# Autodesk Inventor assembly: Assembly3
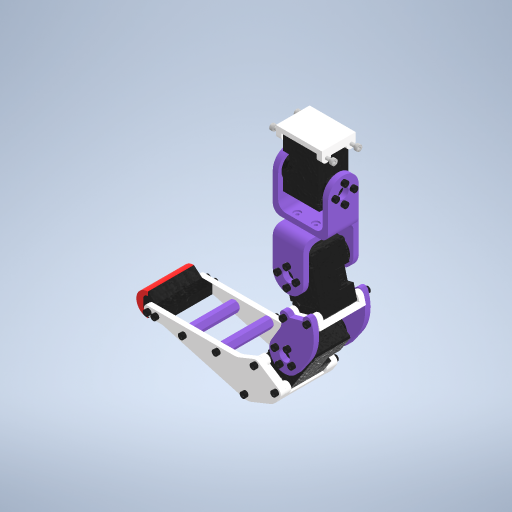
[picture p0: Inventor's stored thumbnail of the model, 512x512]
Saved by Autodesk Inventor 2024 (Build 280153000, 153)
## iProperties
Created: 2024-06-02
Part Number: Assembly3
Document SubType Name: Assembly
Designer: Hemant
Author: Hemant
## iProperties of the stored document DC15_A01_CASE_M_DUMMY.ipt
Created: 2020-07-27
Part Number: DC15_A01_CASE_M_DUMMY
Material: Generic
Description: NOT SPECIFIED
Document SubType Name: Modeling
Designer: Hemant
Mass: 9.54609 g
Surface Area: 36.4084 cm^2
Volume: 9.54609 cm^3
Density: 1 g/cm^3
Appearance: Default
Author: Hemant
Revision Number: 7LAST_VERSION
## iProperties of the stored document PHS_1_7X20_5_DC10.ipt
Created: 2020-07-27
Part Number: PHS_1_7X20_5_DC10
Material: Generic
Description: NOT SPECIFIED
Document SubType Name: Modeling
Designer: Hemant
Density: 1 g/cm^3
Appearance: Default
Author: Hemant
Revision Number: 3LAST_VERSION
## iProperties of the stored document DC15_A01_HORN_DUMMY.ipt
Created: 2020-07-27
Part Number: DC15_A01_HORN_DUMMY
Material: Generic
Description: NOT SPECIFIED
Document SubType Name: Modeling
Designer: Hemant
Density: 1 g/cm^3
Appearance: Default
Author: Hemant
Revision Number: 17LAST_VERSION
## iProperties of the stored document BTS2_M2_6X8.ipt
Created: 2020-07-27
Part Number: BTS2_M2_6X8
Material: Generic
Description: NOT SPECIFIED
Document SubType Name: Modeling
Designer: Hemant
Density: 1 g/cm^3
Appearance: Default
Author: Hemant
Revision Number: 5LAST_VERSION
## iProperties of the stored document DC15_A01_HORN_IDLE2_DUMMY.ipt
Created: 2020-07-27
Part Number: DC15_A01_HORN_IDLE2_DUMMY
Material: Generic
Description: NOT SPECIFIED
Document SubType Name: Modeling
Designer: Hemant
Density: 1 g/cm^3
Appearance: Default
Author: Hemant
Revision Number: 2LAST_VERSION
## iProperties of the stored document XL,XC-330.iam
Created: 2020-07-27
Part Number: DC15_A01_DUMMY_ASSY_IDLE_ASM
Document SubType Name: Assembly
Designer: Hemant
Sending System: CREO PARAMETRIC BY PTC INC, 2019224
Preprocessor: CREO PARAMETRIC BY PTC INC, 2019224
Title: DC15_A01_DUMMY_ASSY_IDLE_ASM
Author: yunever
Revision Number: 9LAST_VERSION
## iProperties of the stored document DC15_A01_CASE_F_DUMMY.ipt
Created: 2020-07-27
Part Number: DC15_A01_CASE_F_DUMMY
Material: Generic
Description: NOT SPECIFIED
Document SubType Name: Modeling
Designer: Hemant
Density: 1 g/cm^3
Appearance: Default
Author: Hemant
Revision Number: 5LAST_VERSION
## iProperties of the stored document DC15_A01_IDLE_CAP_DUMMY.ipt
Created: 2020-07-27
Part Number: DC15_A01_IDLE_CAP_DUMMY
Material: Generic
Description: NOT SPECIFIED
Document SubType Name: Modeling
Designer: Hemant
Density: 1 g/cm^3
Appearance: Default
Author: Hemant
Revision Number: 2LAST_VERSION
## iProperties of the stored document DC15_A01_CASE_B_DUMMY.ipt
Created: 2020-07-27
Part Number: DC15_A01_CASE_B_DUMMY
Material: Generic
Description: NOT SPECIFIED
Document SubType Name: Modeling
Designer: Hemant
Density: 1 g/cm^3
Appearance: Default
Mass: 2.59492 g
Surface Area: 23.2234 cm^2
Volume: 2.59492 cm^3
Author: Hemant
Revision Number: 8LAST_VERSION
## iProperties of the stored document B3B-EH.ipt
Created: 2020-07-27
Part Number: B3B-EH
Material: Generic
Description: NOT SPECIFIED
Document SubType Name: Modeling
Designer: Hemant
Density: 1 g/cm^3
Appearance: Default
Author: Hemant
Revision Number: 2LAST_VERSION
## iProperties of the stored document DC15_A01_LED_CAP2_DUMMY.ipt
Created: 2020-07-27
Part Number: DC15_A01_LED_CAP2_DUMMY
Material: Generic
Description: NOT SPECIFIED
Document SubType Name: Modeling
Designer: Hemant
Density: 1 g/cm^3
Appearance: Default
Author: Hemant
Revision Number: 3LAST_VERSION
## Documents named in this file (22)
- C:\Users\Hemant\Desktop\Studies\MS Proj\V1\Leg_assembly_V2.iam
- **C:\Users\Hemant\Desktop\Studies\MS Proj\V1\Leg_assembly_V2.iam*LocalDocs*xAaaaaedaAaaaaaaaAaaaqztbHd*XL,XC-330.iam
- C:\Users\Hemant\Desktop\Studies\MS Proj\V1\Motor_Bracket.ipt
- C:\Users\Hemant\Desktop\Studies\MS Proj\V1\Motor_Base.ipt
- C:\Users\Hemant\Desktop\Studies\MS Proj\V1\Tibia_Femur_Connect.ipt
- C:\Users\Hemant\Desktop\Studies\MS Proj\V1\Standoff.ipt
- C:\Users\Hemant\Desktop\Studies\MS Proj\V1\socket head cap screw_iso_ISO 4762 M2 x 5 --- 5S.ipt
- C:\Users\Hemant\Desktop\Studies\MS Proj\V1\Tibia_V2.ipt
- C:\Users\Hemant\Desktop\Studies\MS Proj\V1\Foot_V1.ipt
- C:\Users\Hemant\Desktop\Studies\MS Proj\V1\TPU_FootGrip.ipt
- C:\Users\Hemant\Desktop\Studies\MS Proj\XL,XC-330.stp
- **C:\Users\Hemant\Desktop\Studies\MS Proj\V1\Assembly3.iam*LocalDocs*xAaaaaedaAaaaaaaaAaaaqzd4Uh*DC15_A01_CASE_M_DUMMY.ipt
- **C:\Users\Hemant\Desktop\Studies\MS Proj\V1\Assembly3.iam*LocalDocs*xAaaaa1caAaaaaaaaAaaaaeqcGe*PHS_1_7X20_5_DC10.ipt
- **C:\Users\Hemant\Desktop\Studies\MS Proj\V1\Assembly3.iam*LocalDocs*xAaaaa0caAaaaaaaaAaaaan2dPg*DC15_A01_HORN_DUMMY.ipt
- **C:\Users\Hemant\Desktop\Studies\MS Proj\V1\Assembly3.iam*LocalDocs*xAaaaaabaAaaaaaaaAaaaag1aQf*BTS2_M2_6X8.ipt
- **C:\Users\Hemant\Desktop\Studies\MS Proj\V1\Assembly3.iam*LocalDocs*xAaaaalaaAaaaaaaaAaaaqc1fQc*DC15_A01_HORN_IDLE2_DUMMY.ipt
- **C:\Users\Hemant\Desktop\Studies\MS Proj\V1\Assembly3.iam*LocalDocs*xAaaaaedaAaaaaaaaAaaaqztbHd*XL,XC-330.iam
- **C:\Users\Hemant\Desktop\Studies\MS Proj\V1\Assembly3.iam*LocalDocs*xAaaaqebaAaaaaaaaAaaaamr1Rh*DC15_A01_CASE_F_DUMMY.ipt
- **C:\Users\Hemant\Desktop\Studies\MS Proj\V1\Assembly3.iam*LocalDocs*xAaaaqhbaAaaaaaaaAaaaqpykVc*DC15_A01_CASE_B_DUMMY.ipt
- **C:\Users\Hemant\Desktop\Studies\MS Proj\V1\Assembly3.iam*LocalDocs*xAaaaqkcaAaaaaaaaAaaaa1g0If*DC15_A01_LED_CAP2_DUMMY.ipt
- **C:\Users\Hemant\Desktop\Studies\MS Proj\V1\Assembly3.iam*LocalDocs*xAaaaazdaAaaaaaaaAaaaawueFb*DC15_A01_IDLE_CAP_DUMMY.ipt
- **C:\Users\Hemant\Desktop\Studies\MS Proj\V1\Assembly3.iam*LocalDocs*xAaaaqfcaAaaaaaaaAaaaawcvTg*B3B-EH.ipt
## Components (59 placed, 9 different names)
1. XL,XC-330:1 [sub-assembly] — Mate:1, Mate:2_Supress, Mate:3, Mate:4, Mate:5, Mate:6, Angle:3_Supress
2. Motor_Bracket:2 — Mate:1, Mate:2_Supress, Mate:3, Mate:7, Mate:8, Mate:9, Mate:60, Mate:61, Mate:62, Mate:63, Mate:78, Mate:79, Mate:80, Mate:81, Mate:88, Mate:89, Mate:90, Mate:91, Mate:100, Mate:101, Mate:102, Mate:103
3. Motor_Base:1 — Mate:4, Mate:5, Mate:6, Mate:10, Mate:11, Mate:12, Mate:13, Mate:14, Mate:15
4. Motor_Bracket:3 — Mate:7, Mate:8, Mate:9, Mate:16, Mate:17, Mate:26_Supress, Angle:3_Supress, Mate:64, Mate:65, Mate:66, Mate:67, Mate:74, Mate:75, Mate:76, Mate:77
5. Tibia_Femur_Connect:1 — Mate:11, Mate:14, Mate:15, Mate:19, Mate:92, Mate:93, Mate:94, Mate:95, Mate:96, Mate:97, Mate:98, Mate:99, Mate:108, Mate:109, Mate:110, Mate:111
6. Tibia_Femur_Connect:2 — Mate:10, Mate:12, Mate:13, Mate:18, Angle:2_Supress, Mate:56, Mate:57, Mate:58, Mate:59, Mate:70, Mate:71, Mate:72, Mate:73, Mate:84, Mate:85, Mate:86, Mate:87
7. XL,XC-330:2 [sub-assembly] — Mate:16, Mate:17, Angle:1, Mate:26_Supress, Mate:33, Mate:34, Mate:35
8. XL,XC-330:3 [sub-assembly] — Mate:18, Mate:19, Angle:2_Supress, Mate:20, Mate:21, Mate:22
9. Motor_Base:2 — Mate:20, Mate:21, Mate:22, Mate:122, Mate:123, Mate:124, Mate:127, Mate:128, Mate:129
10. Motor_Base:3 — Mate:33, Mate:34, Mate:35, Mate:68, Mate:69, Mate:82, Mate:83, Mate:116, Mate:117, Mate:120, Mate:121, Angle:4_Supress
11. Standoff:1 — Mate:130, Mate:131
12. socket head cap screw_iso_ISO 4762 M2 x 5 --- 5S:2 — Mate:144, Mate:151
13. socket head cap screw_iso_ISO 4762 M2 x 5 --- 5S:3 — Mate:145, Mate:154
14. socket head cap screw_iso_ISO 4762 M2 x 5 --- 5S:4 — Mate:146, Mate:152
15. socket head cap screw_iso_ISO 4762 M2 x 5 --- 5S:5 — Mate:140, Mate:166
16. socket head cap screw_iso_ISO 4762 M2 x 5 --- 5S:6 — Mate:139, Mate:167
17. socket head cap screw_iso_ISO 4762 M2 x 5 --- 5S:7 — Mate:84, Mate:87
18. socket head cap screw_iso_ISO 4762 M2 x 5 --- 5S:8 — Mate:85, Mate:86
19. socket head cap screw_iso_ISO 4762 M2 x 5 --- 5S:9 — Mate:58, Mate:72
20. socket head cap screw_iso_ISO 4762 M2 x 5 --- 5S:10 — Mate:61, Mate:81
21. socket head cap screw_iso_ISO 4762 M2 x 5 --- 5S:11 — Mate:60, Mate:78
22. socket head cap screw_iso_ISO 4762 M2 x 5 --- 5S:12 — Mate:57, Mate:73
23. socket head cap screw_iso_ISO 4762 M2 x 5 --- 5S:13 — Mate:64, Mate:77
24. socket head cap screw_iso_ISO 4762 M2 x 5 --- 5S:14 — Mate:65, Mate:74
25. socket head cap screw_iso_ISO 4762 M2 x 5 --- 5S:15 — Mate:90, Mate:101
26. socket head cap screw_iso_ISO 4762 M2 x 5 --- 5S:16 — Mate:91, Mate:102
27. socket head cap screw_iso_ISO 4762 M2 x 5 --- 5S:17 — Mate:62, Mate:79
28. socket head cap screw_iso_ISO 4762 M2 x 5 --- 5S:18 — Mate:68, Mate:82
29. socket head cap screw_iso_ISO 4762 M2 x 5 --- 5S:19 — Mate:69, Mate:83
30. socket head cap screw_iso_ISO 4762 M2 x 5 --- 5S:20 — Mate:63, Mate:80
31. socket head cap screw_iso_ISO 4762 M2 x 5 --- 5S:21 — Mate:66, Mate:76
32. socket head cap screw_iso_ISO 4762 M2 x 5 --- 5S:22 — Mate:67, Mate:75
33. socket head cap screw_iso_ISO 4762 M2 x 5 --- 5S:23 — Mate:88, Mate:100
34. socket head cap screw_iso_ISO 4762 M2 x 5 --- 5S:24 — Mate:89, Mate:103
35. socket head cap screw_iso_ISO 4762 M2 x 5 --- 5S:25 — Mate:92, Mate:99
36. socket head cap screw_iso_ISO 4762 M2 x 5 --- 5S:26 — Mate:93, Mate:98
37. socket head cap screw_iso_ISO 4762 M2 x 5 --- 5S:27 — Mate:94, Mate:97
38. socket head cap screw_iso_ISO 4762 M2 x 5 --- 5S:28 — Mate:95, Mate:96
39. socket head cap screw_iso_ISO 4762 M2 x 5 --- 5S:30 — Mate:156, Mate:159
40. socket head cap screw_iso_ISO 4762 M2 x 5 --- 5S:31 — Mate:56, Mate:71
41. socket head cap screw_iso_ISO 4762 M2 x 5 --- 5S:32 — Mate:59, Mate:70
42. socket head cap screw_iso_ISO 4762 M2 x 5 --- 5S:35 — Mate:116, Mate:120
43. socket head cap screw_iso_ISO 4762 M2 x 5 --- 5S:36 — Mate:117, Mate:121
44. socket head cap screw_iso_ISO 4762 M2 x 5 --- 5S:37 — Mate:142, Mate:169
45. socket head cap screw_iso_ISO 4762 M2 x 5 --- 5S:38 — Mate:141, Mate:168
46. socket head cap screw_iso_ISO 4762 M2 x 5 --- 5S:39 — Mate:109, Mate:111
47. socket head cap screw_iso_ISO 4762 M2 x 5 --- 5S:40 — Mate:108, Mate:110
48. Tibia_V2:1 — Mate:127, Mate:128, Mate:129, Mate:131, Angle:4_Supress, Mate:137, Mate:139, Mate:140, Mate:144, Mate:145, Mate:146, Mate:151, Mate:152, Mate:154, Mate:166, Mate:167, Mate:171, Mate:172, Mate:178, Mate:179, Mate:180, Mate:181, Angle:5
49. Tibia_V2:2 — Mate:122, Mate:123, Mate:124, Mate:130, Mate:136, Mate:138, Mate:141, Mate:142, Mate:156, Mate:159, Mate:160, Mate:161, Mate:164, Mate:165, Mate:168, Mate:169, Mate:170, Mate:173, Mate:174, Mate:175, Mate:176, Mate:177
50. Foot_V1:1 — Mate:136, Mate:137, Mate:138, Mate:148, Mate:149, Mate:150
51. TPU_FootGrip:1 — Mate:148, Mate:149, Mate:150
52. socket head cap screw_iso_ISO 4762 M2 x 5 --- 5S:41 — Mate:160, Mate:164
53. socket head cap screw_iso_ISO 4762 M2 x 5 --- 5S:42 — Mate:161, Mate:165
54. Standoff:2 — Mate:170, Mate:171, Angle:5
55. socket head cap screw_iso_ISO 4762 M2 x 5 --- 5S:43 — Mate:175, Mate:177
56. socket head cap screw_iso_ISO 4762 M2 x 5 --- 5S:44 — Mate:179, Mate:181
57. Standoff:3 — Mate:172, Mate:173
58. socket head cap screw_iso_ISO 4762 M2 x 5 --- 5S:45 — Mate:174, Mate:176
59. socket head cap screw_iso_ISO 4762 M2 x 5 --- 5S:46 — Mate:178, Mate:180
## Relationships (133: Mate 128, Angle 5)
- Mate:1: XL,XC-330:1 ↔ Motor_Bracket:2
- Mate:2_Supress: XL,XC-330:1 ↔ Motor_Bracket:2
- Mate:3: XL,XC-330:1 ↔ Motor_Bracket:2
- Mate:4: XL,XC-330:1 ↔ Motor_Base:1
- Mate:5: XL,XC-330:1 ↔ Motor_Base:1
- Mate:6: XL,XC-330:1 ↔ Motor_Base:1
- Mate:7: Motor_Bracket:2 ↔ Motor_Bracket:3
- Mate:8: Motor_Bracket:2 ↔ Motor_Bracket:3
- Mate:9: Motor_Bracket:2 ↔ Motor_Bracket:3
- Mate:10: Motor_Base:1 ↔ Tibia_Femur_Connect:2
- Mate:11: Motor_Base:1 ↔ Tibia_Femur_Connect:1
- Mate:12: Motor_Base:1 ↔ Tibia_Femur_Connect:2
- Mate:13: Motor_Base:1 ↔ Tibia_Femur_Connect:2
- Mate:14: Motor_Base:1 ↔ Tibia_Femur_Connect:1
- Mate:15: Motor_Base:1 ↔ Tibia_Femur_Connect:1
- Mate:16: Motor_Bracket:3 ↔ XL,XC-330:2
- Mate:17: Motor_Bracket:3 ↔ XL,XC-330:2
- Angle:1 (0 deg): XL,XC-330:2
- Mate:18: Tibia_Femur_Connect:2 ↔ XL,XC-330:3
- Mate:19 (0.5 mm): Tibia_Femur_Connect:1 ↔ XL,XC-330:3
- Angle:2_Supress (0 deg): Tibia_Femur_Connect:2 ↔ XL,XC-330:3
- Mate:20: XL,XC-330:3 ↔ Motor_Base:2
- Mate:21: XL,XC-330:3 ↔ Motor_Base:2
- Mate:22: XL,XC-330:3 ↔ Motor_Base:2
- Mate:26_Supress: Motor_Bracket:3 ↔ XL,XC-330:2
- Angle:3_Supress (0 deg): XL,XC-330:1 ↔ Motor_Bracket:3
- Mate:33: XL,XC-330:2 ↔ Motor_Base:3
- Mate:34: XL,XC-330:2 ↔ Motor_Base:3
- Mate:35: XL,XC-330:2 ↔ Motor_Base:3
- Mate:56: Tibia_Femur_Connect:2 ↔ socket head cap screw_iso_ISO 4762 M2 x 5 --- 5S:31
- Mate:57: Tibia_Femur_Connect:2 ↔ socket head cap screw_iso_ISO 4762 M2 x 5 --- 5S:12
- Mate:58: Tibia_Femur_Connect:2 ↔ socket head cap screw_iso_ISO 4762 M2 x 5 --- 5S:9
- Mate:59: Tibia_Femur_Connect:2 ↔ socket head cap screw_iso_ISO 4762 M2 x 5 --- 5S:32
- Mate:60: Motor_Bracket:2 ↔ socket head cap screw_iso_ISO 4762 M2 x 5 --- 5S:11
- Mate:61: Motor_Bracket:2 ↔ socket head cap screw_iso_ISO 4762 M2 x 5 --- 5S:10
- Mate:62: Motor_Bracket:2 ↔ socket head cap screw_iso_ISO 4762 M2 x 5 --- 5S:17
- Mate:63: Motor_Bracket:2 ↔ socket head cap screw_iso_ISO 4762 M2 x 5 --- 5S:20
- Mate:64: Motor_Bracket:3 ↔ socket head cap screw_iso_ISO 4762 M2 x 5 --- 5S:13
- Mate:65: Motor_Bracket:3 ↔ socket head cap screw_iso_ISO 4762 M2 x 5 --- 5S:14
- Mate:66: Motor_Bracket:3 ↔ socket head cap screw_iso_ISO 4762 M2 x 5 --- 5S:21
- Mate:67: Motor_Bracket:3 ↔ socket head cap screw_iso_ISO 4762 M2 x 5 --- 5S:22
- Mate:68 (3.5 mm): Motor_Base:3 ↔ socket head cap screw_iso_ISO 4762 M2 x 5 --- 5S:18
- Mate:69 (3.5 mm): Motor_Base:3 ↔ socket head cap screw_iso_ISO 4762 M2 x 5 --- 5S:19
- Mate:70: Tibia_Femur_Connect:2 ↔ socket head cap screw_iso_ISO 4762 M2 x 5 --- 5S:32
- Mate:71: Tibia_Femur_Connect:2 ↔ socket head cap screw_iso_ISO 4762 M2 x 5 --- 5S:31
- Mate:72: Tibia_Femur_Connect:2 ↔ socket head cap screw_iso_ISO 4762 M2 x 5 --- 5S:9
- Mate:73: Tibia_Femur_Connect:2 ↔ socket head cap screw_iso_ISO 4762 M2 x 5 --- 5S:12
- Mate:74: Motor_Bracket:3 ↔ socket head cap screw_iso_ISO 4762 M2 x 5 --- 5S:14
- Mate:75: Motor_Bracket:3 ↔ socket head cap screw_iso_ISO 4762 M2 x 5 --- 5S:22
- Mate:76: Motor_Bracket:3 ↔ socket head cap screw_iso_ISO 4762 M2 x 5 --- 5S:21
- Mate:77: Motor_Bracket:3 ↔ socket head cap screw_iso_ISO 4762 M2 x 5 --- 5S:13
- Mate:78: Motor_Bracket:2 ↔ socket head cap screw_iso_ISO 4762 M2 x 5 --- 5S:11
- Mate:79: Motor_Bracket:2 ↔ socket head cap screw_iso_ISO 4762 M2 x 5 --- 5S:17
- Mate:80: Motor_Bracket:2 ↔ socket head cap screw_iso_ISO 4762 M2 x 5 --- 5S:20
- Mate:81: Motor_Bracket:2 ↔ socket head cap screw_iso_ISO 4762 M2 x 5 --- 5S:10
- Mate:82: Motor_Base:3 ↔ socket head cap screw_iso_ISO 4762 M2 x 5 --- 5S:18
- Mate:83: Motor_Base:3 ↔ socket head cap screw_iso_ISO 4762 M2 x 5 --- 5S:19
- Mate:84: Tibia_Femur_Connect:2 ↔ socket head cap screw_iso_ISO 4762 M2 x 5 --- 5S:7
- Mate:85: Tibia_Femur_Connect:2 ↔ socket head cap screw_iso_ISO 4762 M2 x 5 --- 5S:8
- Mate:86: Tibia_Femur_Connect:2 ↔ socket head cap screw_iso_ISO 4762 M2 x 5 --- 5S:8
- Mate:87: Tibia_Femur_Connect:2 ↔ socket head cap screw_iso_ISO 4762 M2 x 5 --- 5S:7
- Mate:88: Motor_Bracket:2 ↔ socket head cap screw_iso_ISO 4762 M2 x 5 --- 5S:23
- Mate:89: Motor_Bracket:2 ↔ socket head cap screw_iso_ISO 4762 M2 x 5 --- 5S:24
- Mate:90: Motor_Bracket:2 ↔ socket head cap screw_iso_ISO 4762 M2 x 5 --- 5S:15
- Mate:91: Motor_Bracket:2 ↔ socket head cap screw_iso_ISO 4762 M2 x 5 --- 5S:16
- Mate:92: Tibia_Femur_Connect:1 ↔ socket head cap screw_iso_ISO 4762 M2 x 5 --- 5S:25
- Mate:93: Tibia_Femur_Connect:1 ↔ socket head cap screw_iso_ISO 4762 M2 x 5 --- 5S:26
- Mate:94: Tibia_Femur_Connect:1 ↔ socket head cap screw_iso_ISO 4762 M2 x 5 --- 5S:27
- Mate:95: Tibia_Femur_Connect:1 ↔ socket head cap screw_iso_ISO 4762 M2 x 5 --- 5S:28
- Mate:96: Tibia_Femur_Connect:1 ↔ socket head cap screw_iso_ISO 4762 M2 x 5 --- 5S:28
- Mate:97: Tibia_Femur_Connect:1 ↔ socket head cap screw_iso_ISO 4762 M2 x 5 --- 5S:27
- Mate:98: Tibia_Femur_Connect:1 ↔ socket head cap screw_iso_ISO 4762 M2 x 5 --- 5S:26
- Mate:99: Tibia_Femur_Connect:1 ↔ socket head cap screw_iso_ISO 4762 M2 x 5 --- 5S:25
- Mate:100: Motor_Bracket:2 ↔ socket head cap screw_iso_ISO 4762 M2 x 5 --- 5S:23
- Mate:101: Motor_Bracket:2 ↔ socket head cap screw_iso_ISO 4762 M2 x 5 --- 5S:15
- Mate:102: Motor_Bracket:2 ↔ socket head cap screw_iso_ISO 4762 M2 x 5 --- 5S:16
- Mate:103: Motor_Bracket:2 ↔ socket head cap screw_iso_ISO 4762 M2 x 5 --- 5S:24
- Mate:108: Tibia_Femur_Connect:1 ↔ socket head cap screw_iso_ISO 4762 M2 x 5 --- 5S:40
- Mate:109: Tibia_Femur_Connect:1 ↔ socket head cap screw_iso_ISO 4762 M2 x 5 --- 5S:39
- Mate:110: Tibia_Femur_Connect:1 ↔ socket head cap screw_iso_ISO 4762 M2 x 5 --- 5S:40
- Mate:111: Tibia_Femur_Connect:1 ↔ socket head cap screw_iso_ISO 4762 M2 x 5 --- 5S:39
- Mate:116 (3.5 mm): Motor_Base:3 ↔ socket head cap screw_iso_ISO 4762 M2 x 5 --- 5S:35
- Mate:117 (3.5 mm): Motor_Base:3 ↔ socket head cap screw_iso_ISO 4762 M2 x 5 --- 5S:36
- Mate:120: Motor_Base:3 ↔ socket head cap screw_iso_ISO 4762 M2 x 5 --- 5S:35
- Mate:121: Motor_Base:3 ↔ socket head cap screw_iso_ISO 4762 M2 x 5 --- 5S:36
- Mate:122: Motor_Base:2 ↔ Tibia_V2:2
- Mate:123: Motor_Base:2 ↔ Tibia_V2:2
- Mate:124: Motor_Base:2 ↔ Tibia_V2:2
- Mate:127: Motor_Base:2 ↔ Tibia_V2:1
- Mate:128: Motor_Base:2 ↔ Tibia_V2:1
- Mate:129: Motor_Base:2 ↔ Tibia_V2:1
- Mate:130: Standoff:1 ↔ Tibia_V2:2
- Mate:131: Standoff:1 ↔ Tibia_V2:1
- Angle:4_Supress (0 deg): Motor_Base:3 ↔ Tibia_V2:1
- Mate:136: Tibia_V2:2 ↔ Foot_V1:1
- Mate:137: Tibia_V2:1 ↔ Foot_V1:1
- Mate:138: Tibia_V2:2 ↔ Foot_V1:1
- Mate:139: socket head cap screw_iso_ISO 4762 M2 x 5 --- 5S:6 ↔ Tibia_V2:1
- Mate:140: socket head cap screw_iso_ISO 4762 M2 x 5 --- 5S:5 ↔ Tibia_V2:1
- Mate:141: socket head cap screw_iso_ISO 4762 M2 x 5 --- 5S:38 ↔ Tibia_V2:2
- Mate:142: socket head cap screw_iso_ISO 4762 M2 x 5 --- 5S:37 ↔ Tibia_V2:2
- Mate:144: socket head cap screw_iso_ISO 4762 M2 x 5 --- 5S:2 ↔ Tibia_V2:1
- Mate:145: socket head cap screw_iso_ISO 4762 M2 x 5 --- 5S:3 ↔ Tibia_V2:1
- Mate:146: socket head cap screw_iso_ISO 4762 M2 x 5 --- 5S:4 ↔ Tibia_V2:1
- Mate:148: Foot_V1:1 ↔ TPU_FootGrip:1
- Mate:149: Foot_V1:1 ↔ TPU_FootGrip:1
- Mate:150: Foot_V1:1 ↔ TPU_FootGrip:1
- Mate:151: socket head cap screw_iso_ISO 4762 M2 x 5 --- 5S:2 ↔ Tibia_V2:1
- Mate:152: socket head cap screw_iso_ISO 4762 M2 x 5 --- 5S:4 ↔ Tibia_V2:1
- Mate:154: socket head cap screw_iso_ISO 4762 M2 x 5 --- 5S:3 ↔ Tibia_V2:1
- Mate:156: socket head cap screw_iso_ISO 4762 M2 x 5 --- 5S:30 ↔ Tibia_V2:2
- Mate:159: socket head cap screw_iso_ISO 4762 M2 x 5 --- 5S:30 ↔ Tibia_V2:2
- Mate:160: Tibia_V2:2 ↔ socket head cap screw_iso_ISO 4762 M2 x 5 --- 5S:41
- Mate:161: Tibia_V2:2 ↔ socket head cap screw_iso_ISO 4762 M2 x 5 --- 5S:42
- Mate:164: Tibia_V2:2 ↔ socket head cap screw_iso_ISO 4762 M2 x 5 --- 5S:41
- Mate:165: Tibia_V2:2 ↔ socket head cap screw_iso_ISO 4762 M2 x 5 --- 5S:42
- Mate:166: socket head cap screw_iso_ISO 4762 M2 x 5 --- 5S:5 ↔ Tibia_V2:1
- Mate:167: socket head cap screw_iso_ISO 4762 M2 x 5 --- 5S:6 ↔ Tibia_V2:1
- Mate:168: socket head cap screw_iso_ISO 4762 M2 x 5 --- 5S:38 ↔ Tibia_V2:2
- Mate:169: socket head cap screw_iso_ISO 4762 M2 x 5 --- 5S:37 ↔ Tibia_V2:2
- Mate:170: Tibia_V2:2 ↔ Standoff:2
- Mate:171: Tibia_V2:1 ↔ Standoff:2
- Mate:172: Tibia_V2:1 ↔ Standoff:3
- Mate:173: Tibia_V2:2 ↔ Standoff:3
- Mate:174: Tibia_V2:2 ↔ socket head cap screw_iso_ISO 4762 M2 x 5 --- 5S:45
- Mate:175: Tibia_V2:2 ↔ socket head cap screw_iso_ISO 4762 M2 x 5 --- 5S:43
- Mate:176: Tibia_V2:2 ↔ socket head cap screw_iso_ISO 4762 M2 x 5 --- 5S:45
- Mate:177: Tibia_V2:2 ↔ socket head cap screw_iso_ISO 4762 M2 x 5 --- 5S:43
- Mate:178: Tibia_V2:1 ↔ socket head cap screw_iso_ISO 4762 M2 x 5 --- 5S:46
- Mate:179: Tibia_V2:1 ↔ socket head cap screw_iso_ISO 4762 M2 x 5 --- 5S:44
- Mate:180: Tibia_V2:1 ↔ socket head cap screw_iso_ISO 4762 M2 x 5 --- 5S:46
- Mate:181: Tibia_V2:1 ↔ socket head cap screw_iso_ISO 4762 M2 x 5 --- 5S:44
- Angle:5 (0 deg): Tibia_V2:1 ↔ Standoff:2
